# Autodesk Inventor assembly: Throughput Mockup Assembly
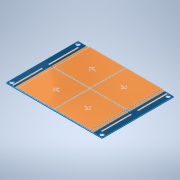
[picture p0: Inventor's stored thumbnail of the model, 180x180]
Saved by Autodesk Inventor 2022 (Build 260153000, 153)
## iProperties
Created: 2022-04-25
Part Number: Throughput Mockup Assembly
Document SubType Name: Assembly
Designer: Caleb
Author: Caleb
## iProperties of the stored document coppers_fuse#F.Cu.ipt
Created: 2022-05-02
Part Number: coppers_fuse#F.Cu
Material: Generic
Document SubType Name: Modeling
Designer: Caleb
Density: 1 g/cm^3
Appearance: Default
Author: Caleb
## iProperties of the stored document etl_module_pcb_mockup_v3.iam
Created: 2022-04-25
Part Number: etl_module_pcb_mockup_v3
Description: FreeCAD Model
Document SubType Name: Assembly
Designer: Caleb
Authority: Unknown
Sending System: FreeCAD
Preprocessor: Open CASCADE STEP processor 7.5
Title: Open CASCADE Shape Model
Author: Author
## iProperties of the stored document board_solid.ipt
Created: 2022-05-02
Part Number: board_solid
Material: Generic
Document SubType Name: Modeling
Designer: Caleb
Density: 1 g/cm^3
Appearance: Default
Author: Caleb
## Documents named in this file (7)
- C:\Users\Caleb\Desktop\nebraska-silicon-lab\Hardware\ETL\modules\throughput mockups\Throughput Mockup Assembly.iam
- **C:\Users\Caleb\Desktop\nebraska-silicon-lab\Hardware\ETL\modules\throughput mockups\Throughput Mockup Assembly.iam*LocalDocs*xAaaaa3aaAaaaaaaaAaaaqdqrQh*etl_module_pcb_mockup_v3.iam
- C:\Users\Caleb\Desktop\nebraska-silicon-lab\Hardware\ETL\modules\throughput mockups\BBM Assembly.iam
- C:\Users\Caleb\Desktop\nebraska-silicon-lab\Hardware\ETL\ETL-SH-Design\3D-model\K3D-WP7B-S050VA1-V3_JAE_Proprietary v1_14.iam
- **C:\Users\Caleb\Desktop\nebraska-silicon-lab\Hardware\ETL\modules\throughput mockups\Throughput Mockup Assembly.iam*LocalDocs*xAaaaq0baAaaaaaaaAaaaqqhp2c*coppers_fuse#F.Cu.ipt
- **C:\Users\Caleb\Desktop\nebraska-silicon-lab\Hardware\ETL\modules\throughput mockups\Throughput Mockup Assembly.iam*LocalDocs*xAaaaq2daAaaaaaaaAaaaqb5oDc*board_solid.ipt
- C:\Users\Caleb\Desktop\nebraska-silicon-lab\Hardware\ETL\modules\throughput mockups\etl_module_pcb_mockup_v3.step
## Components (7 placed, 3 different names)
1. etl_module_pcb_mockup_v3:1 [sub-assembly] — Mate:1, Mate:2, Mate:3, Mate:4, Angle:1, Angle:2, Angle:3, Angle:4, Flush:5, Flush:6, Mate:7, Mate:8
2. BBM Assembly:1 [sub-assembly] — Mate:1, Angle:2, Mate:5, Flush:1, Mate:6, Flush:2
3. BBM Assembly:2 [sub-assembly] — Mate:3, Angle:4, Mate:6, Flush:2, Flush:3
4. BBM Assembly:3 [sub-assembly] — Mate:4, Angle:3, Flush:3, Flush:4, Flush:6
5. BBM Assembly:4 [sub-assembly] — Mate:2, Angle:1, Mate:5, Flush:1, Flush:4, Flush:5
6. K3D-WP7B-S050VA1-V3_JAE_Proprietary v1_14:1 [sub-assembly] — Mate:7
7. K3D-WP7B-S050VA1-V3_JAE_Proprietary v1_14:2 [sub-assembly] — Mate:8
## Relationships (18: Mate 8, Flush 6, Angle 4)
- Mate:1: etl_module_pcb_mockup_v3:1 ↔ BBM Assembly:1
- Mate:2: etl_module_pcb_mockup_v3:1 ↔ BBM Assembly:4
- Mate:3: etl_module_pcb_mockup_v3:1 ↔ BBM Assembly:2
- Mate:4: etl_module_pcb_mockup_v3:1 ↔ BBM Assembly:3
- Angle:1 (0 deg): etl_module_pcb_mockup_v3:1 ↔ BBM Assembly:4
- Angle:2 (0 deg): etl_module_pcb_mockup_v3:1 ↔ BBM Assembly:1
- Angle:3 (0 deg): etl_module_pcb_mockup_v3:1 ↔ BBM Assembly:3
- Angle:4 (0 deg): etl_module_pcb_mockup_v3:1 ↔ BBM Assembly:2
- Mate:5 (0.2 mm): BBM Assembly:1 ↔ BBM Assembly:4
- Flush:1: BBM Assembly:1 ↔ BBM Assembly:4
- Mate:6 (0.2 mm): BBM Assembly:1 ↔ BBM Assembly:2
- Flush:2: BBM Assembly:1 ↔ BBM Assembly:2
- Flush:3: BBM Assembly:2 ↔ BBM Assembly:3
- Flush:4: BBM Assembly:3 ↔ BBM Assembly:4
- Flush:5 (0.05 mm): etl_module_pcb_mockup_v3:1 ↔ BBM Assembly:4
- Flush:6 (5.45 mm): etl_module_pcb_mockup_v3:1 ↔ BBM Assembly:3
- Mate:7: etl_module_pcb_mockup_v3:1 ↔ K3D-WP7B-S050VA1-V3_JAE_Proprietary v1_14:1
- Mate:8: etl_module_pcb_mockup_v3:1 ↔ K3D-WP7B-S050VA1-V3_JAE_Proprietary v1_14:2
